# Autodesk Inventor assembly: SklopReduktora
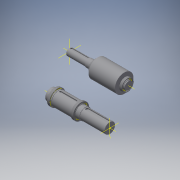
[picture p0: Inventor's stored thumbnail of the model, 180x180]
Saved by Autodesk Inventor 2018 (Build 220112000, 112)
## iProperties
Created: 2018-11-17
Part Number: SklopReduktora
Document SubType Name: Assembly
Designer: Kristijan
Author: Kristijan
## Documents named in this file (5)
- C:\Users\Kristijan\Dropbox\PolitehnikaPula\5 semestar\Konstrukcije\TimskiProjektniZadatak\OutputDrawings\SklopReduktora.iam
- C:\Users\Kristijan\Dropbox\PolitehnikaPula\5 semestar\Konstrukcije\TimskiProjektniZadatak\OutputDrawings\PogonskoVratilo.ipt
- C:\Users\Kristijan\Dropbox\PolitehnikaPula\5 semestar\Konstrukcije\TimskiProjektniZadatak\datasheetsModels\6008.iam
- C:\Users\Kristijan\Dropbox\PolitehnikaPula\5 semestar\Konstrukcije\TimskiProjektniZadatak\OutputDrawings\GonjenoVratilo.ipt
- C:\Users\Kristijan\Dropbox\PolitehnikaPula\5 semestar\Konstrukcije\TimskiProjektniZadatak\datasheetsModels\32913.iam
## Components (6 placed, 4 different names)
1. PogonskoVratilo:1 — Mate:1, Mate:3, Mate:4, Mate:5, Mate:10, Mate:12
2. 6008:1 [sub-assembly] — Mate:3, Mate:4
3. 6008:2 [sub-assembly] — Mate:1, Mate:5, Flush:14
4. GonjenoVratilo:1 — Mate:6, Mate:7, Mate:8, Mate:9, Mate:11
5. 32913:1 [sub-assembly] — Mate:6, Mate:7, Flush:14
6. 32913:2 [sub-assembly] — Mate:8, Mate:9
## Relationships (12: Mate 11, Flush 1)
- Mate:1: PogonskoVratilo:1 ↔ 6008:2
- Mate:3: PogonskoVratilo:1 ↔ 6008:1
- Mate:4: PogonskoVratilo:1 ↔ 6008:1
- Mate:5: PogonskoVratilo:1 ↔ 6008:2
- Mate:6: GonjenoVratilo:1 ↔ 32913:1
- Mate:7: GonjenoVratilo:1 ↔ 32913:1
- Mate:8: GonjenoVratilo:1 ↔ 32913:2
- Mate:9: GonjenoVratilo:1 ↔ 32913:2
- Mate:10: PogonskoVratilo:1
- Mate:11 (264.5 mm): GonjenoVratilo:1
- Mate:12: PogonskoVratilo:1
- Flush:14: 6008:2 ↔ 32913:1
